# Autodesk Inventor assembly: HbthumbU01
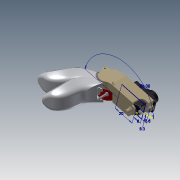
[picture p0: Inventor's stored thumbnail of the model, 180x180]
Saved by Autodesk Inventor 2015 SP1 (Build 190203100, 203)
## iProperties
Created: 2015-02-19
Part Number: HbthumbU01
Document SubType Name: Assembly
Designer: Yamaura
Author: Yamaura
## Documents named in this file (8)
- C:\Users\Yamaura\Documents\GitHub\HACKberry\HACKberry-hardware\3D\Inventor\Parts\HbthumbU01.iam
- C:\Users\Yamaura\Documents\GitHub\HACKberry\HACKberry-hardware\3D\Inventor\Parts\ASV-15MG.ipt
- C:\Users\Yamaura\Documents\GitHub\HACKberry\HACKberry-hardware\3D\Inventor\Parts\ScrewM2L8.ipt
- C:\Users\Yamaura\Documents\GitHub\HACKberry\HACKberry-hardware\3D\Inventor\Parts\HbThumbLockButton01.ipt
- C:\Users\Yamaura\Documents\GitHub\HACKberry\HACKberry-hardware\3D\Inventor\Parts\HbThumbProximalPhalanx01.ipt
- C:\Users\Yamaura\Documents\GitHub\HACKberry\HACKberry-hardware\3D\Inventor\Parts\HbThumbMetacarpalPhalanx01.ipt
- C:\Users\Yamaura\Documents\GitHub\HACKberry\HACKberry-hardware\3D\Inventor\Parts\HbThumbMetacarpalPhalanxCover01.ipt
- C:\Users\Yamaura\Documents\GitHub\HACKberry\HACKberry-hardware\3D\Inventor\Parts\CP 0.5-6-8.ipt
## Components (9 placed, 7 different names)
1. ASV-15MG:1 — メイト:27, メイト:28, メイト:29
2. ScrewM2L8:1
3. ScrewM2L8:2
4. HbThumbLockButton01:1 — メイト:31, メイト:32, 角度:5
5. HbThumbMetacarpalPhalanx01:1 — メイト:21, 角度:4, フラッシュ:3, メイト:26, メイト:27, メイト:28, メイト:29, メイト:30, メイト:32, メイト:33
6. HbThumbMetacarpalPhalanxCover01:1 — メイト:24, メイト:30, メイト:33
7. CP 0.5-6-8:1 — メイト:25, メイト:26
8. HbThumbProximalPhalanx01:1 — メイト:19, メイト:20
9. HbThumbProximalPhalanx01:2
## Component patterns: (2 elements, first: HbThumbProximalPhalanx01:1)
## Relationships (16: Mate 13, Angle 2, Flush 1)
- メイト:19 [Mate] (-1.5 mm): HbThumbProximalPhalanx01:1
- メイト:20 [Mate]: HbThumbProximalPhalanx01:1
- メイト:21 [Mate]: HbThumbMetacarpalPhalanx01:1
- 角度:4 [Angle] (0 deg): HbThumbMetacarpalPhalanx01:1
- フラッシュ:3 [Flush] (9.5 mm): HbThumbMetacarpalPhalanx01:1
- メイト:24 [Mate]: HbThumbMetacarpalPhalanxCover01:1
- メイト:25 [Mate]: CP 0.5-6-8:1
- メイト:26 [Mate]: HbThumbMetacarpalPhalanx01:1 ↔ CP 0.5-6-8:1
- メイト:27 [Mate]: ASV-15MG:1 ↔ HbThumbMetacarpalPhalanx01:1
- メイト:28 [Mate]: ASV-15MG:1 ↔ HbThumbMetacarpalPhalanx01:1
- メイト:29 [Mate]: ASV-15MG:1 ↔ HbThumbMetacarpalPhalanx01:1
- メイト:30 [Mate]: HbThumbMetacarpalPhalanx01:1 ↔ HbThumbMetacarpalPhalanxCover01:1
- メイト:31 [Mate]: HbThumbLockButton01:1
- メイト:32 [Mate] (2 mm): HbThumbLockButton01:1 ↔ HbThumbMetacarpalPhalanx01:1
- 角度:5 [Angle] (40 deg): HbThumbLockButton01:1
- メイト:33 [Mate]: HbThumbMetacarpalPhalanx01:1 ↔ HbThumbMetacarpalPhalanxCover01:1
